# Autodesk Inventor assembly: Z Motor Assembly
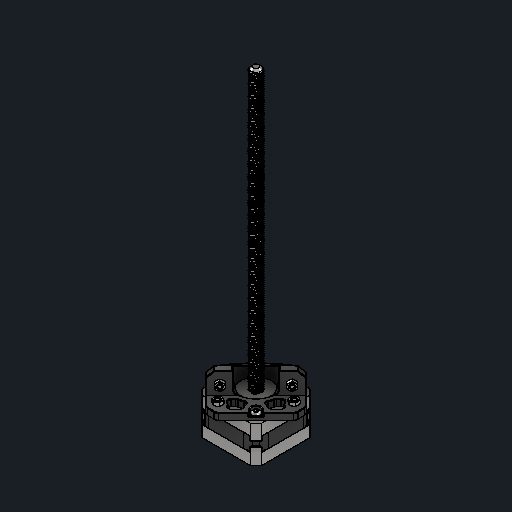
[picture p0: Inventor's stored thumbnail of the model, 512x512]
Saved by Autodesk Inventor 2026.1 (Build 301233020, 233B)
## iProperties
Created: 2025-05-09
Part Number: Z Motor Assembly
Document SubType Name: Assembly
Designer: AdminForWorker
Title: Z Motor Assembly
Author: AdminForWorker
## Documents named in this file (5)
- C:\Users\JoshuaEah\Documents\GitHub\Voron-0\CAD\Z Axis\Z Motor Assembly.iam
- C:\Users\JoshuaEah\Documents\GitHub\Voron-0\CAD\Z Axis\Parts\200mm Integrated Leadscrew Stepper.ipt
- C:\Users\JoshuaEah\Documents\GitHub\Voron-0\CAD\Z Axis\Parts\Z Motor Mount.ipt
- C:\Users\JoshuaEah\Documents\GitHub\Voron-0\CAD\Hardware\M3x8 BHCS.ipt
- C:\Users\JoshuaEah\Documents\GitHub\Voron-0\CAD\Hardware\M3 Hexnut.ipt
## Components (13 placed, 4 different names)
1. 200mm Integrated Leadscrew Stepper:1 — Insert:8, Insert:9
2. Z Motor Mount:1 — Insert:1, Insert:2, Mate:1, Mate:2, Insert:7, Mate:3, Insert:8, Insert:9, Insert:10
3. M3x8 BHCS:1 — Insert:1
4. M3x8 BHCS:2 — Insert:6, Insert:7
5. M3x8 BHCS:3 — Mate:1
6. M3x8 BHCS:4 — Insert:2, Insert:3
7. M3x8 BHCS:5 — Mate:2, Insert:4
8. M3x8 BHCS:6 — Insert:5, Mate:3
9. M3x8 BHCS:7 — Insert:10
10. M3 Hexnut:1 — Insert:5
11. M3 Hexnut:2 — Insert:4
12. M3 Hexnut:3 — Insert:6
13. M3 Hexnut:4 — Insert:3
## Relationships (13: Insert 10, Mate 3)
- Insert:1: Z Motor Mount:1 ↔ M3x8 BHCS:1
- Insert:2: Z Motor Mount:1 ↔ M3x8 BHCS:4
- Mate:1: Z Motor Mount:1 ↔ M3x8 BHCS:3
- Mate:2: Z Motor Mount:1 ↔ M3x8 BHCS:5
- Insert:3: M3x8 BHCS:4 ↔ M3 Hexnut:4
- Insert:4: M3x8 BHCS:5 ↔ M3 Hexnut:2
- Insert:5: M3x8 BHCS:6 ↔ M3 Hexnut:1
- Insert:6: M3x8 BHCS:2 ↔ M3 Hexnut:3
- Insert:7: Z Motor Mount:1 ↔ M3x8 BHCS:2
- Mate:3: Z Motor Mount:1 ↔ M3x8 BHCS:6
- Insert:8: 200mm Integrated Leadscrew Stepper:1 ↔ Z Motor Mount:1
- Insert:9: 200mm Integrated Leadscrew Stepper:1 ↔ Z Motor Mount:1
- Insert:10: Z Motor Mount:1 ↔ M3x8 BHCS:7
